# Autodesk Inventor assembly: driver_ass_1
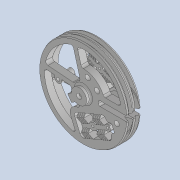
[picture p0: Inventor's stored thumbnail of the model, 180x180]
Saved by Autodesk Inventor 2020 (Build 240168000, 168)
## iProperties
Created: 2021-07-20
Part Number: driver_ass_1
Document SubType Name: Assembly
Designer: Shuang Peng
Author: Shuang Peng
## Documents named in this file (2)
- D:\projects-3\torque fb tip\hardware\tip_2\driver_ass_1.iam
- D:\projects-3\torque fb tip\hardware\tip_2\driver_wheel_1.ipt
## Components (2 placed, 1 different names)
1. driver_wheel_1:1 — Flush:1, Insert:1
2. driver_wheel_1:2 — Flush:1, Insert:1
## Relationships (2: Flush 1, Insert 1)
- Flush:1: driver_wheel_1:1 ↔ driver_wheel_1:2
- Insert:1: driver_wheel_1:1 ↔ driver_wheel_1:2
